# Autodesk Inventor assembly: Assembly
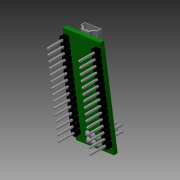
[picture p0: Inventor's stored thumbnail of the model, 180x180]
Saved by Autodesk Inventor 2015 (Build 190159000, 159)
## iProperties
Created: 2015-09-08
Part Number: Assembly
Document SubType Name: Weldment
Designer: david
Weld Material: Aluminum 6061, Welded
Author: david
## Documents named in this file (8)
- Z:\gip\generatie 6\frame\bak\electronica\Arduino nano\Assembly.iam
- Z:\gip\generatie 6\frame\bak\electronica\Arduino nano\bord.ipt
- Z:\gip\generatie 6\frame\bak\electronica\Arduino nano\staafje.ipt
- Z:\gip\generatie 6\frame\bak\electronica\Arduino nano\USB-slot.ipt
- Z:\gip\generatie 6\frame\bak\electronica\Arduino nano\2.ipt
- Z:\gip\generatie 6\frame\bak\electronica\Arduino nano\knop_1.ipt
- Z:\gip\generatie 6\frame\bak\electronica\Arduino nano\led.ipt
- Z:\gip\generatie 6\frame\bak\electronica\Arduino nano\block.ipt
## Components (80 placed, 7 different names)
1. bord:1 — Mate:1, Flush:1, Mate:2, Flush:2, Flush:3, Mate:3, Mate:5, Mate:6, Flush:4, Mate:8, Mate:9, Mate:10, Mate:11, Flush:8, Mate:16, Mate:17, Mate:18, Mate:19, Mate:20, Mate:21, Flush:9, Flush:10, Flush:11, Flush:12, Flush:13, Flush:14, Angle:2, Mate:23, Mate:25, Angle:3
2. USB-slot:1 — Mate:2, Flush:2, Flush:3, Mate:4, Angle:1
3. 2:1 — Mate:3, Mate:4, Angle:1, Mate:5, Mate:7
4. knop_1:1 — Mate:6, Flush:4, Mate:7, Mate:15
5. led:1 — Mate:8, Flush:5, Mate:14, Flush:8, Mate:15
6. led:2 — Mate:10, Flush:5, Flush:6, Mate:13, Mate:14
7. led:3 — Mate:9, Flush:7, Mate:12
8. led:4 — Mate:11, Flush:6, Flush:7, Mate:12, Mate:13
9. staafje:31 — Mate:16, Flush:11
10. staafje:32 — Mate:18, Flush:10
11. staafje:33 — Mate:17, Flush:12
12. staafje:34 — Mate:19, Flush:14, Mate:22
13. staafje:35 — Mate:20, Flush:13
14. staafje:36 — Mate:21, Flush:9
15. staafje:1 — Mate:1, Flush:1
16. staafje:2
17. staafje:3
18. staafje:4
19. staafje:5
20. staafje:6
21. staafje:7
22. staafje:8
23. staafje:9
24. staafje:10
25. staafje:11
26. staafje:12
27. staafje:13
28. staafje:14
29. staafje:15
30. staafje:16
31. staafje:17
32. staafje:18
33. staafje:19
34. staafje:20
35. staafje:21
36. staafje:22
37. staafje:23
38. staafje:24
39. staafje:25
40. staafje:26
41. staafje:27
42. staafje:28
43. staafje:29 — Mate:24
44. staafje:30
45. block:1 — Mate:22, Angle:2, Mate:23
46. block:2
47. block:3
48. block:4
49. block:5
50. block:6
51. block:7 — Mate:24, Mate:25, Angle:3
52. block:8
53. block:9
54. block:10
55. block:11
56. block:12
57. block:13
58. block:14
59. block:15
60. block:16
61. block:17
62. block:18
63. block:19
64. block:20
65. block:21
66. block:22
67. block:23
68. block:24
69. block:25
70. block:26
71. block:27
72. block:28
73. block:29
74. block:30
75. block:31
76. block:32
77. block:33
78. block:34
79. block:35
80. block:36
## Component patterns: (30 elements, first: staafje:1), (6 elements, first: block:1), (30 elements, first: block:7)
## Relationships (42: Mate 25, Flush 14, Angle 3)
- Mate:1: bord:1 ↔ staafje:1
- Flush:1 (-1 mm): bord:1 ↔ staafje:1
- Mate:2: bord:1 ↔ USB-slot:1
- Flush:2 (5 mm): bord:1 ↔ USB-slot:1
- Flush:3 (-1 mm): bord:1 ↔ USB-slot:1
- Mate:3: bord:1 ↔ 2:1
- Mate:4 (3 mm): USB-slot:1 ↔ 2:1
- Angle:1 (135 deg): USB-slot:1 ↔ 2:1
- Mate:5 (-4 mm): bord:1 ↔ 2:1
- Mate:6: bord:1 ↔ knop_1:1
- Flush:4 (7 mm): bord:1 ↔ knop_1:1
- Mate:7 (2 mm): 2:1 ↔ knop_1:1
- Mate:8: bord:1 ↔ led:1
- Mate:9: bord:1 ↔ led:3
- Mate:10: bord:1 ↔ led:2
- Mate:11: bord:1 ↔ led:4
- Flush:5: led:1 ↔ led:2
- Flush:6: led:2 ↔ led:4
- Flush:7: led:3 ↔ led:4
- Mate:12 (1.5 mm): led:3 ↔ led:4
- Mate:13 (1.5 mm): led:2 ↔ led:4
- Mate:14 (1.5 mm): led:1 ↔ led:2
- Flush:8 (4.75 mm): bord:1 ↔ led:1
- Mate:15 (1.5 mm): knop_1:1 ↔ led:1
- Mate:16: bord:1 ↔ staafje:31
- Mate:17: bord:1 ↔ staafje:33
- Mate:18: bord:1 ↔ staafje:32
- Mate:19: bord:1 ↔ staafje:34
- Mate:20: bord:1 ↔ staafje:35
- Mate:21: bord:1 ↔ staafje:36
- Flush:9 (-1 mm): bord:1 ↔ staafje:36
- Flush:10 (-1 mm): bord:1 ↔ staafje:32
- Flush:11 (1 mm): bord:1 ↔ staafje:31
- Flush:12 (-1 mm): bord:1 ↔ staafje:33
- Flush:13 (-1 mm): bord:1 ↔ staafje:35
- Flush:14 (-1 mm): bord:1 ↔ staafje:34
- Mate:22: staafje:34 ↔ block:1
- Angle:2 (0 deg): bord:1 ↔ block:1
- Mate:23: bord:1 ↔ block:1
- Mate:24: staafje:29 ↔ block:7
- Mate:25: bord:1 ↔ block:7
- Angle:3 (0 deg): bord:1 ↔ block:7
